# Autodesk Inventor assembly: Moving platform and legs
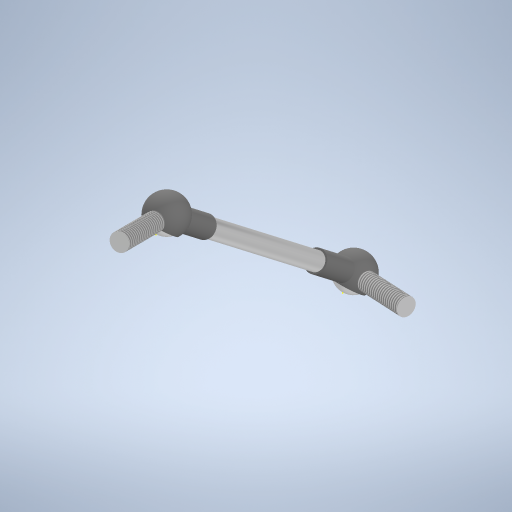
[picture p0: Inventor's stored thumbnail of the model, 512x512]
Saved by Autodesk Inventor 2023 (Build 270158000, 158)
## iProperties
Created: 2022-06-29
Part Number: Moving platform and legs
Document SubType Name: Assembly
Designer: earls
Author: earls
## Documents named in this file (4)
- F:\Documents\Mechatronic Engineering 5.1\Project\CAD\Moving platform and legs.iam
- F:\Documents\Mechatronic Engineering 5.1\Project\CAD\Rod qty-6.ipt
- F:\Documents\Mechatronic Engineering 5.1\Project\CAD\Spherical joint\Part1.ipt
- F:\Documents\Mechatronic Engineering 5.1\Project\CAD\Spherical joint\Part2.ipt
## Components (5 placed, 3 different names)
1. Rod qty-6:1 — Rotational:1, Rotational:2
2. Part1:1 — Rotational:1, Ball:1
3. Part2:1 — Ball:1
4. Part1:2 — Rotational:2, Ball:2
5. Part2:2 — Ball:2
## Relationships (4: RevoluteJoint 2, BallJoint 2)
- Rotational:1 [RevoluteJoint]: Rod qty-6:1 ↔ Part1:1
- Ball:1: Part1:1 ↔ Part2:1
- Rotational:2 [RevoluteJoint]: Rod qty-6:1 ↔ Part1:2
- Ball:2: Part1:2 ↔ Part2:2
